# Autodesk Inventor assembly: Laufkatze_Baugruppe
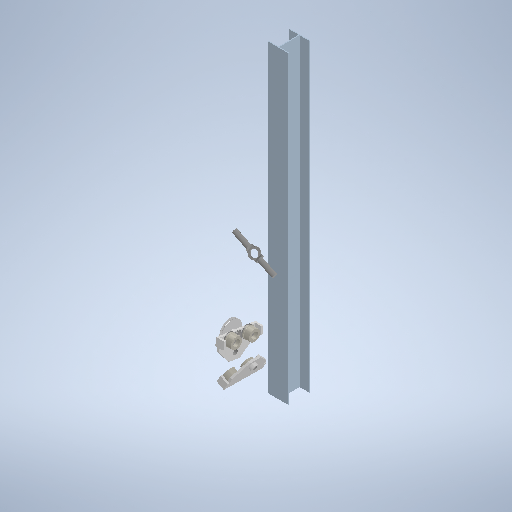
[picture p0: Inventor's stored thumbnail of the model, 512x512]
Saved by Autodesk Inventor 2025.2 (Build 292293000, 293)
## iProperties
Created: 2025-02-03
Part Number: Laufkatze_Baugruppe
Document SubType Name: Assembly
Designer: unter
Author: unter
## Documents named in this file (15)
- C:\Users\unter\OneDrive\Desktop\Uni\03_WS2025\Advanced_Mechanical_Engeneering_2\Konstruktion\Projekt\Laufkatze\Baugruppen\Laufkatze_Baugruppe.iam
- C:\Users\unter\OneDrive\Desktop\Uni\03_WS2025\Advanced_Mechanical_Engeneering_2\Konstruktion\Projekt\Laufkatze\Einzelbauteile\Stahlträger.ipt
- C:\Users\unter\OneDrive\Desktop\Uni\03_WS2025\Advanced_Mechanical_Engeneering_2\Konstruktion\Projekt\Laufkatze\Einzelbauteile\Führungsplatte_links.ipt
- C:\Users\unter\OneDrive\Desktop\Uni\03_WS2025\Advanced_Mechanical_Engeneering_2\Konstruktion\Projekt\Laufkatze\Einzelbauteile\Laufrad.ipt
- C:\Users\unter\OneDrive\Desktop\Uni\03_WS2025\Advanced_Mechanical_Engeneering_2\Konstruktion\Projekt\Laufkatze\Baugruppen\Laufkatze_Baugruppe\Konstruktions-Assistent\Lager1.iam
- C:\Users\unter\OneDrive\Desktop\Uni\03_WS2025\Advanced_Mechanical_Engeneering_2\Konstruktion\Projekt\Laufkatze\Einzelbauteile\Führungsplatte_rechts.ipt
- C:\Users\unter\OneDrive\Desktop\Uni\03_WS2025\Advanced_Mechanical_Engeneering_2\Konstruktion\Projekt\Laufkatze\Einzelbauteile\Zahnrad_bei_Laufrad.ipt
- C:\Users\unter\OneDrive\Desktop\Uni\03_WS2025\Advanced_Mechanical_Engeneering_2\Konstruktion\Projekt\Laufkatze\Einzelbauteile\Welle_für_Kettenzug.ipt
- C:\Users\unter\OneDrive\Desktop\Uni\03_WS2025\Advanced_Mechanical_Engeneering_2\Konstruktion\Projekt\Laufkatze\Baugruppen\Laufkatze_Baugruppe\Konstruktions-Assistent\Lager4.iam
- C:\Users\unter\OneDrive\Desktop\Uni\03_WS2025\Advanced_Mechanical_Engeneering_2\Konstruktion\Projekt\Laufkatze\Einzelbauteile\Zahnrad_für_Kettenzug.ipt
- C:\Users\unter\OneDrive\Desktop\Uni\03_WS2025\Advanced_Mechanical_Engeneering_2\Konstruktion\Projekt\Laufkatze\Einzelbauteile\Zugscheibe_für_Kette.ipt
- C:\Users\unter\OneDrive\Desktop\Uni\03_WS2025\Advanced_Mechanical_Engeneering_2\Konstruktion\Projekt\Laufkatze\Einzelbauteile\Schraubbolzen.ipt
- C:\Users\unter\OneDrive\Desktop\Uni\03_WS2025\Advanced_Mechanical_Engeneering_2\Konstruktion\Projekt\Laufkatze\Normteile\de-DE\DIN EN ISO 7093-2\DIN EN ISO 7093-2 - 12.ipt
- C:\Users\unter\OneDrive\Desktop\Uni\03_WS2025\Advanced_Mechanical_Engeneering_2\Konstruktion\Projekt\Laufkatze\Normteile\de-DE\DIN EN ISO 7093-2\DIN EN ISO 7093-2 - 14.ipt
- C:\Users\unter\OneDrive\Desktop\Uni\03_WS2025\Advanced_Mechanical_Engeneering_2\Konstruktion\Projekt\Laufkatze\Normteile\de-DE\ISO 8676(1)\ISO 8676 - M12 x 1,25 x 30DIN EN.ipt
## Components (31 placed, 13 different names)
1. Stahlträger:1
2. Führungsplatte_links:1 — Passend:1, Passend:3, Passend:4, Passend:5, Passend:45, Passend:46
3. Laufrad:1 — Passend:1, Passend:4, Passend:8, Passend:9, Passend:41
4. Laufrad:2 — Passend:3, Passend:5, Passend:6, Passend:7, Passend:42
5. Lager:1 [sub-assembly] — Passend:8, Passend:9, Passend:43
6. Lager:2 [sub-assembly] — Passend:6, Passend:7, Passend:44
7. Führungsplatte_rechts:1 — Passend:14, Passend:15, Passend:16, Passend:17, Passend:22, Passend:23, Passend:24, Passend:30, Passend:32, Passend:33, Passend:35, Passend:49, Passend:50
8. Laufrad:3 — Passend:10, Passend:11, Passend:20, Passend:38
9. Laufrad:4 — Passend:12, Passend:13, Passend:14, Passend:21, Passend:37
10. Zahnrad_bei_Laufrad:1 — Passend:10, Passend:11, Passend:16, Passend:17
11. Zahnrad_bei_Laufrad:2 — Passend:12, Passend:13, Passend:15
12. Lager:3 [sub-assembly] — Passend:20, Passend:23, Passend:40
13. Lager:4 [sub-assembly] — Passend:21, Passend:22, Passend:39
14. Welle_für_Kettenzug:1 — Passend:24, Passend:25, Passend:26, Passend:27, Passend:28, Passend:29, Fluchtend:1, Passend:31, Fluchtend:2, Passend:34, Passend:36, Passend:53, Passend:55
15. Lager:5 [sub-assembly] — Passend:25, Passend:26
16. Lager:6 [sub-assembly] — Passend:27, Passend:28
17. Zahnrad_für_Kettenzug:1 — Passend:29, Fluchtend:1, Passend:30
18. Zugscheibe_für_Kette:1 — Passend:31, Fluchtend:2
19. Schraubbolzen:1
20. DIN EN ISO 7093-2 12:1 — Passend:32, Passend:33, Passend:34, Passend:54
21. DIN EN ISO 7093-2 12:2 — Passend:35, Passend:36, Passend:56
22. DIN EN ISO 7093-2 14:1 — Passend:37, Passend:39, Passend:51
23. DIN EN ISO 7093-2 14:2 — Passend:38, Passend:40, Passend:52
24. DIN EN ISO 7093-2 14:3 — Passend:41, Passend:43, Passend:47
25. DIN EN ISO 7093-2 14:4 — Passend:42, Passend:44, Passend:48
26. DIN EN 28676 M12 x 1,25 x 30:1 — Passend:45, Passend:47
27. DIN EN 28676 M12 x 1,25 x 30:2 — Passend:46, Passend:48
28. DIN EN 28676 M12 x 1,25 x 30:3 — Passend:49, Passend:51
29. DIN EN 28676 M12 x 1,25 x 30:4 — Passend:50, Passend:52
30. DIN EN 28676 M12 x 1,25 x 30:5 — Passend:53, Passend:54
31. DIN EN 28676 M12 x 1,25 x 30:6 — Passend:55, Passend:56
## Relationships (55: Mate 53, Flush 2)
- Passend:1 [Mate]: Führungsplatte_links:1 ↔ Laufrad:1
- Passend:3 [Mate]: Führungsplatte_links:1 ↔ Laufrad:2
- Passend:4 [Mate] (2 mm): Führungsplatte_links:1 ↔ Laufrad:1
- Passend:5 [Mate] (2 mm): Führungsplatte_links:1 ↔ Laufrad:2
- Passend:6 [Mate]: Laufrad:2 ↔ Lager:2
- Passend:7 [Mate]: Laufrad:2 ↔ Lager:2
- Passend:8 [Mate]: Laufrad:1 ↔ Lager:1
- Passend:9 [Mate]: Laufrad:1 ↔ Lager:1
- Passend:10 [Mate]: Laufrad:3 ↔ Zahnrad_bei_Laufrad:1
- Passend:11 [Mate]: Laufrad:3 ↔ Zahnrad_bei_Laufrad:1
- Passend:12 [Mate]: Laufrad:4 ↔ Zahnrad_bei_Laufrad:2
- Passend:13 [Mate]: Laufrad:4 ↔ Zahnrad_bei_Laufrad:2
- Passend:14 [Mate]: Führungsplatte_rechts:1 ↔ Laufrad:4
- Passend:15 [Mate] (2 mm): Führungsplatte_rechts:1 ↔ Zahnrad_bei_Laufrad:2
- Passend:16 [Mate]: Führungsplatte_rechts:1 ↔ Zahnrad_bei_Laufrad:1
- Passend:17 [Mate] (2 mm): Führungsplatte_rechts:1 ↔ Zahnrad_bei_Laufrad:1
- Passend:20 [Mate]: Laufrad:3 ↔ Lager:3
- Passend:21 [Mate]: Laufrad:4 ↔ Lager:4
- Passend:22 [Mate]: Führungsplatte_rechts:1 ↔ Lager:4
- Passend:23 [Mate]: Führungsplatte_rechts:1 ↔ Lager:3
- Passend:24 [Mate]: Führungsplatte_rechts:1 ↔ Welle_für_Kettenzug:1
- Passend:25 [Mate]: Welle_für_Kettenzug:1 ↔ Lager:5
- Passend:26 [Mate]: Welle_für_Kettenzug:1 ↔ Lager:5
- Passend:27 [Mate]: Welle_für_Kettenzug:1 ↔ Lager:6
- Passend:28 [Mate]: Welle_für_Kettenzug:1 ↔ Lager:6
- Passend:29 [Mate]: Welle_für_Kettenzug:1 ↔ Zahnrad_für_Kettenzug:1
- Fluchtend:1 [Flush]: Welle_für_Kettenzug:1 ↔ Zahnrad_für_Kettenzug:1
- Passend:30 [Mate] (2 mm): Führungsplatte_rechts:1 ↔ Zahnrad_für_Kettenzug:1
- Passend:31 [Mate]: Welle_für_Kettenzug:1 ↔ Zugscheibe_für_Kette:1
- Fluchtend:2 [Flush]: Welle_für_Kettenzug:1 ↔ Zugscheibe_für_Kette:1
- Passend:32 [Mate]: Führungsplatte_rechts:1 ↔ DIN EN ISO 7093-2 12:1
- Passend:33 [Mate]: Führungsplatte_rechts:1 ↔ DIN EN ISO 7093-2 12:1
- Passend:34 [Mate]: Welle_für_Kettenzug:1 ↔ DIN EN ISO 7093-2 12:1
- Passend:35 [Mate]: Führungsplatte_rechts:1 ↔ DIN EN ISO 7093-2 12:2
- Passend:36 [Mate]: Welle_für_Kettenzug:1 ↔ DIN EN ISO 7093-2 12:2
- Passend:37 [Mate]: Laufrad:4 ↔ DIN EN ISO 7093-2 14:1
- Passend:38 [Mate]: Laufrad:3 ↔ DIN EN ISO 7093-2 14:2
- Passend:39 [Mate]: Lager:4 ↔ DIN EN ISO 7093-2 14:1
- Passend:40 [Mate]: Lager:3 ↔ DIN EN ISO 7093-2 14:2
- Passend:41 [Mate]: Laufrad:1 ↔ DIN EN ISO 7093-2 14:3
- Passend:42 [Mate]: Laufrad:2 ↔ DIN EN ISO 7093-2 14:4
- Passend:43 [Mate]: Lager:1 ↔ DIN EN ISO 7093-2 14:3
- Passend:44 [Mate]: Lager:2 ↔ DIN EN ISO 7093-2 14:4
- Passend:45 [Mate]: Führungsplatte_links:1 ↔ DIN EN 28676 M12 x 1,25 x 30:1
- Passend:46 [Mate]: Führungsplatte_links:1 ↔ DIN EN 28676 M12 x 1,25 x 30:2
- Passend:47 [Mate]: DIN EN ISO 7093-2 14:3 ↔ DIN EN 28676 M12 x 1,25 x 30:1
- Passend:48 [Mate]: DIN EN ISO 7093-2 14:4 ↔ DIN EN 28676 M12 x 1,25 x 30:2
- Passend:49 [Mate]: Führungsplatte_rechts:1 ↔ DIN EN 28676 M12 x 1,25 x 30:3
- Passend:50 [Mate]: Führungsplatte_rechts:1 ↔ DIN EN 28676 M12 x 1,25 x 30:4
- Passend:51 [Mate]: DIN EN ISO 7093-2 14:1 ↔ DIN EN 28676 M12 x 1,25 x 30:3
- Passend:52 [Mate]: DIN EN ISO 7093-2 14:2 ↔ DIN EN 28676 M12 x 1,25 x 30:4
- Passend:53 [Mate]: Welle_für_Kettenzug:1 ↔ DIN EN 28676 M12 x 1,25 x 30:5
- Passend:54 [Mate]: DIN EN ISO 7093-2 12:1 ↔ DIN EN 28676 M12 x 1,25 x 30:5
- Passend:55 [Mate]: Welle_für_Kettenzug:1 ↔ DIN EN 28676 M12 x 1,25 x 30:6
- Passend:56 [Mate]: DIN EN ISO 7093-2 12:2 ↔ DIN EN 28676 M12 x 1,25 x 30:6
